# Autodesk Inventor assembly: Microcontroller_board_Nano_square
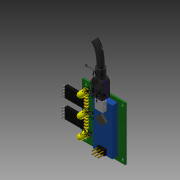
[picture p0: Inventor's stored thumbnail of the model, 180x180]
Saved by Autodesk Inventor 2016 (Build 200138000, 138)
## iProperties
Created: 2015-06-12
Part Number: Microcontroller_board_Nano_square
Document SubType Name: Assembly
Designer: Openlab
Author: Openlab
## Documents named in this file (5)
- D:\Alexey\HS-Spectrophotometer\parts\Common\Microcontroller_board_Nano_square.iam
- D:\Alexey\HS-Spectrophotometer\parts\Common\Pin-connector-angled-4.iam
- D:\Alexey\HS-Spectrophotometer\parts\Common\LED.ipt
- D:\Alexey\HS-Spectrophotometer\parts\Common\Mini_USB_cable.ipt
- D:\Alexey\HS-Spectrophotometer\parts\Common\Microcontroller_board_Nano_square.ipt
## Components (7 placed, 4 different names)
1. Pin-connector-angled-4:1 [sub-assembly] — Mate:2, Mate:4, Mate:5
2. Pin-connector-angled-4:2 [sub-assembly] — Mate:1, Mate:3, Mate:6
3. LED:1 — Mate:9, Mate:10
4. LED:2 — Mate:7, Mate:8
5. LED:3 — Mate:11, Mate:12
6. Mini_USB_cable:1 — Mate:13, Mate:14, Mate:15
7. Microcontroller_board_Nano_square:1 — Mate:1, Mate:2, Mate:3, Mate:4, Mate:5, Mate:6, Mate:7, Mate:8, Mate:9, Mate:10, Mate:11, Mate:12, Mate:13, Mate:14, Mate:15
## Relationships (15: Mate 15)
- Mate:1: Pin-connector-angled-4:2 ↔ Microcontroller_board_Nano_square:1
- Mate:2: Pin-connector-angled-4:1 ↔ Microcontroller_board_Nano_square:1
- Mate:3: Pin-connector-angled-4:2 ↔ Microcontroller_board_Nano_square:1
- Mate:4: Pin-connector-angled-4:1 ↔ Microcontroller_board_Nano_square:1
- Mate:5: Pin-connector-angled-4:1 ↔ Microcontroller_board_Nano_square:1
- Mate:6: Pin-connector-angled-4:2 ↔ Microcontroller_board_Nano_square:1
- Mate:7: LED:2 ↔ Microcontroller_board_Nano_square:1
- Mate:8: LED:2 ↔ Microcontroller_board_Nano_square:1
- Mate:9: LED:1 ↔ Microcontroller_board_Nano_square:1
- Mate:10: LED:1 ↔ Microcontroller_board_Nano_square:1
- Mate:11: LED:3 ↔ Microcontroller_board_Nano_square:1
- Mate:12: LED:3 ↔ Microcontroller_board_Nano_square:1
- Mate:13: Mini_USB_cable:1 ↔ Microcontroller_board_Nano_square:1
- Mate:14: Mini_USB_cable:1 ↔ Microcontroller_board_Nano_square:1
- Mate:15: Mini_USB_cable:1 ↔ Microcontroller_board_Nano_square:1
